# Autodesk Inventor assembly: Motor_MainAxis_Assembly
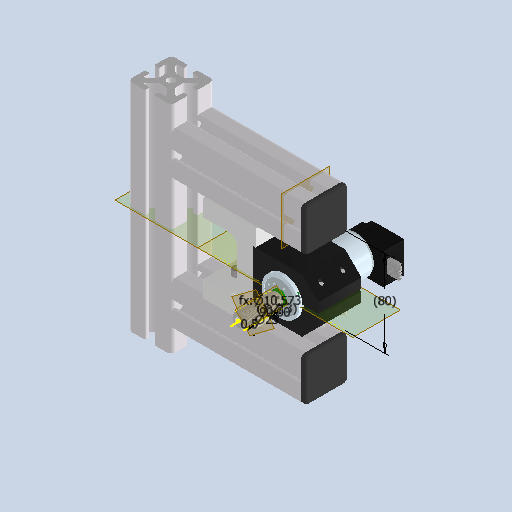
[picture p0: Inventor's stored thumbnail of the model, 512x512]
Saved by Autodesk Inventor 2024 (Build 280153000, 153)
## iProperties
Created: 2022-07-26
Part Number: Motor_MainAxis_Assembly
Document SubType Name: Assembly
Designer: alexw
Motor_Frame_FixationPlate_Width: 80.000 mm
Author: alexw
## Documents named in this file (14)
- C:\Users\AEWALDER\Documents\Inventor\03_CurrentProjects\MasterThesis\PSM_V1_Rillenkugellager\Motor_MainAxis_Assembly.iam
- C:\Users\AEWALDER\Documents\Inventor\03_CurrentProjects\MasterThesis\PSM_V1_Rillenkugellager\Motor_MainAxis_Fixation_Holder.ipt
- C:\Users\AEWALDER\Documents\Inventor\03_CurrentProjects\MasterThesis\PSM_V1_Rillenkugellager\273752_RE35_GB_90W_KL_2WE.ipt
- C:\Users\AEWALDER\Documents\Inventor\03_CurrentProjects\MasterThesis\PSM_V1_Rillenkugellager\Drehbuchse.ipt
- C:\Users\AEWALDER\Documents\Inventor\03_CurrentProjects\MasterThesis\PSM_V1_Rillenkugellager\Item_200_Bodenquerverbindung.ipt
- C:\Users\AEWALDER\Documents\Inventor\03_CurrentProjects\MasterThesis\PSM_V1_Rillenkugellager\Motor_MainAxis_Frame_Fixation.ipt
- C:\Users\AEWALDER\Documents\Inventor\03_CurrentProjects\MasterThesis\PSM_V1_Rillenkugellager\Item_MotorFrame_Strebe.ipt
- C:\Users\AEWALDER\Documents\Inventor\03_CurrentProjects\MasterThesis\PSM_V1_Rillenkugellager\Maschinenbauteil\item_0049433_abdeckkappe_profil_st_8_40x40_details_3.ipt
- C:\Users\AEWALDER\Documents\Inventor\03_CurrentProjects\MasterThesis\PSM_V1_Rillenkugellager\Capstonradialdisc.ipt
- C:\Users\AEWALDER\Documents\Inventor\03_CurrentProjects\MasterThesis\PSM_V1_Rillenkugellager\ContentCenter\de-DE\ISO 4762(2)\ISO 4762 - M5 x 25ISO.ipt
- C:\Users\AEWALDER\Documents\Inventor\03_CurrentProjects\MasterThesis\PSM_V1_Rillenkugellager\ContentCenter\de-DE\ISO 4762(2)\ISO 4762 - M4 x 25ISO.ipt
- C:\Users\AEWALDER\Documents\Inventor\03_CurrentProjects\MasterThesis\PSM_V1_Rillenkugellager\ContentCenter\de-DE\ISO 4762(2)\ISO 4762 - M4 x 30ISO.ipt
- C:\Users\AEWALDER\Documents\Inventor\03_CurrentProjects\MasterThesis\PSM_V1_Rillenkugellager\AVAGO_HEDS_5540_A1.ipt
- C:\Users\AEWALDER\Documents\Inventor\03_CurrentProjects\MasterThesis\PSM_V1_Rillenkugellager\Capston_Drive_Motorwelle.ipt
## Components (16 placed, 11 different names)
1. Motor_MainAxis_Fixation_Holder:1 — Passend:8, Passend:20, Passend:21, Passend:22, Passend:23, Passend:24, Passend:25, Passend:26, Winkel:2
2. 273752_RE35_GB_90W_KL_2WE:1 — Passend:8, Passend:31, Passend:41, Passend:42, Mate:43, Mate:44
3. Capston_Drive_Motorwelle:1 — Mate:43, Mate:44
4. Item_200_Bodenquerverbindung:1 — Passend:13, Fluchtend:6, Fluchtend:7, Passend:14, Fluchtend:8, Fluchtend:9, Passend:15, Fluchtend:11
5. Item_MotorFrame_Strebe:1 — Passend:13, Fluchtend:6, Fluchtend:7, Symmetrie:1, Passend:27, Passend:28, Winkel:1
6. Item_MotorFrame_Strebe:2 — Passend:14, Fluchtend:8, Fluchtend:9, Passend:17, Symmetrie:1, Passend:19, Fluchtend:10, Passend:29, Passend:30
7. Motor_MainAxis_Frame_Fixation:1 — Passend:19, Fluchtend:10, Passend:20, Passend:21, Passend:22, Passend:33, Passend:34, Passend:35, Passend:36, Passend:37, Passend:38, Passend:39, Passend:40
8. ISO 4762 M4 x 30:2 — Passend:23, Passend:24
9. ISO 4762 M4 x 30:1 — Passend:25, Passend:26
10. item_0049433_abdeckkappe_profil_st_8_40x40_details_3:1 — Passend:29, Passend:30
11. item_0049433_abdeckkappe_profil_st_8_40x40_details_3:2 — Passend:27, Passend:28
12. ISO 4762 M5 x 25:1 — Passend:33, Passend:34
13. ISO 4762 M5 x 25:2 — Passend:35, Passend:36
14. ISO 4762 M4 x 25:1 — Passend:37, Passend:38
15. ISO 4762 M4 x 25:2 — Passend:39, Passend:40
16. AVAGO_HEDS_5540_A1:1 — Passend:41, Winkel:2, Passend:42
## Relationships (41: Mate 32, Flush 6, Angle 2, Symmetry 1)
- Passend:8 [Mate]: Motor_MainAxis_Fixation_Holder:1 ↔ 273752_RE35_GB_90W_KL_2WE:1
- Passend:13 [Mate]: Item_200_Bodenquerverbindung:1 ↔ Item_MotorFrame_Strebe:1
- Fluchtend:6 [Flush] (20 mm): Item_200_Bodenquerverbindung:1 ↔ Item_MotorFrame_Strebe:1
- Fluchtend:7 [Flush]: Item_200_Bodenquerverbindung:1 ↔ Item_MotorFrame_Strebe:1
- Passend:14 [Mate]: Item_200_Bodenquerverbindung:1 ↔ Item_MotorFrame_Strebe:2
- Fluchtend:8 [Flush] (20 mm): Item_200_Bodenquerverbindung:1 ↔ Item_MotorFrame_Strebe:2
- Fluchtend:9 [Flush]: Item_200_Bodenquerverbindung:1 ↔ Item_MotorFrame_Strebe:2
- Passend:15 [Mate]: Item_200_Bodenquerverbindung:1
- Passend:17 [Mate]: Item_MotorFrame_Strebe:2
- Symmetrie:1: Item_MotorFrame_Strebe:1 ↔ Item_MotorFrame_Strebe:2
- Passend:18 [Mate]
- Passend:19 [Mate]: Item_MotorFrame_Strebe:2 ↔ Motor_MainAxis_Frame_Fixation:1
- Fluchtend:10 [Flush]: Item_MotorFrame_Strebe:2 ↔ Motor_MainAxis_Frame_Fixation:1
- Passend:20 [Mate]: Motor_MainAxis_Fixation_Holder:1 ↔ Motor_MainAxis_Frame_Fixation:1
- Passend:21 [Mate]: Motor_MainAxis_Fixation_Holder:1 ↔ Motor_MainAxis_Frame_Fixation:1
- Passend:22 [Mate]: Motor_MainAxis_Fixation_Holder:1 ↔ Motor_MainAxis_Frame_Fixation:1
- Passend:23 [Mate]: Motor_MainAxis_Fixation_Holder:1 ↔ ISO 4762 M4 x 30:2
- Passend:24 [Mate]: Motor_MainAxis_Fixation_Holder:1 ↔ ISO 4762 M4 x 30:2
- Passend:25 [Mate]: Motor_MainAxis_Fixation_Holder:1 ↔ ISO 4762 M4 x 30:1
- Passend:26 [Mate]: Motor_MainAxis_Fixation_Holder:1 ↔ ISO 4762 M4 x 30:1
- Passend:27 [Mate]: Item_MotorFrame_Strebe:1 ↔ item_0049433_abdeckkappe_profil_st_8_40x40_details_3:2
- Passend:28 [Mate]: Item_MotorFrame_Strebe:1 ↔ item_0049433_abdeckkappe_profil_st_8_40x40_details_3:2
- Passend:29 [Mate]: Item_MotorFrame_Strebe:2 ↔ item_0049433_abdeckkappe_profil_st_8_40x40_details_3:1
- Passend:30 [Mate]: Item_MotorFrame_Strebe:2 ↔ item_0049433_abdeckkappe_profil_st_8_40x40_details_3:1
- Passend:31 [Mate]: 273752_RE35_GB_90W_KL_2WE:1
- Passend:32 [Mate]
- Winkel:1 [Angle] (90 deg): Item_MotorFrame_Strebe:1
- Fluchtend:11 [Flush] (-104 mm): Item_200_Bodenquerverbindung:1
- Passend:33 [Mate]: Motor_MainAxis_Frame_Fixation:1 ↔ ISO 4762 M5 x 25:1
- Passend:34 [Mate]: Motor_MainAxis_Frame_Fixation:1 ↔ ISO 4762 M5 x 25:1
- Passend:35 [Mate]: Motor_MainAxis_Frame_Fixation:1 ↔ ISO 4762 M5 x 25:2
- Passend:36 [Mate]: Motor_MainAxis_Frame_Fixation:1 ↔ ISO 4762 M5 x 25:2
- Passend:37 [Mate]: Motor_MainAxis_Frame_Fixation:1 ↔ ISO 4762 M4 x 25:1
- Passend:38 [Mate]: Motor_MainAxis_Frame_Fixation:1 ↔ ISO 4762 M4 x 25:1
- Passend:39 [Mate]: Motor_MainAxis_Frame_Fixation:1 ↔ ISO 4762 M4 x 25:2
- Passend:40 [Mate]: Motor_MainAxis_Frame_Fixation:1 ↔ ISO 4762 M4 x 25:2
- Passend:41 [Mate]: 273752_RE35_GB_90W_KL_2WE:1 ↔ AVAGO_HEDS_5540_A1:1
- Winkel:2 [Angle] (0 deg): Motor_MainAxis_Fixation_Holder:1 ↔ AVAGO_HEDS_5540_A1:1
- Passend:42 [Mate]: 273752_RE35_GB_90W_KL_2WE:1 ↔ AVAGO_HEDS_5540_A1:1
- Mate:43: 273752_RE35_GB_90W_KL_2WE:1 ↔ Capston_Drive_Motorwelle:1
- Mate:44: 273752_RE35_GB_90W_KL_2WE:1 ↔ Capston_Drive_Motorwelle:1
## Named parameters: Motor_Frame_FixationPlate_Width = 80 mm, CapstonBig_Radius = 120 mm, BigCaptson_DrivePart_Dia = 12 mm
